# Autodesk Inventor assembly: POM_T5_31
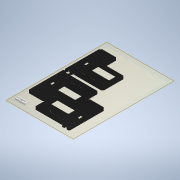
[picture p0: Inventor's stored thumbnail of the model, 180x180]
Saved by Autodesk Inventor 2020 (Build 240168000, 168)
## iProperties
Created: 2021-08-27
Part Number: POM_T5_31
Document SubType Name: Assembly
Designer: Masato
Author: Masato
## Documents named in this file (5)
- D:\GitHub\inventor\SUSTAINA-OP\Cam\POM_T5_31.iam
- D:\GitHub\inventor\SUSTAINA-OP\Cam\DisposableBoard.ipt
- D:\GitHub\inventor\SUSTAINA-OP\Jig\ForeArm_diagonal_Jig_2.ipt
- D:\GitHub\inventor\SUSTAINA-OP\UpperBody\Cockpit\Cockpit_side_frame.ipt
- D:\GitHub\inventor\SUSTAINA-OP\UpperBody\Cockpit\Cockpit_side_frame_MIR.ipt
## Components (5 placed, 4 different names)
1. DisposableBoard:1 — メイト:2, メイト:1, フラッシュ:1, フラッシュ:2, メイト:4, メイト:5, メイト:14, メイト:16, メイト:17, メイト:18, メイト:22, メイト:23, メイト:25
2. ForeArm_diagonal_Jig_2:1 — メイト:14, メイト:16, メイト:23
3. Cockpit_side_frame:1 — メイト:4, メイト:24, メイト:25
4. Cockpit_side_frame_MIR:2 — メイト:5, メイト:20, メイト:21, メイト:22, メイト:24
5. Cockpit_side_frame_MIR:3 — メイト:17, メイト:18, メイト:20, メイト:21
## Relationships (16: Mate 14, Flush 2)
- メイト:2 [Mate]: DisposableBoard:1
- メイト:1 [Mate]: DisposableBoard:1
- フラッシュ:1 [Flush]: DisposableBoard:1
- フラッシュ:2 [Flush]: DisposableBoard:1
- メイト:4 [Mate]: DisposableBoard:1 ↔ Cockpit_side_frame:1
- メイト:5 [Mate]: DisposableBoard:1 ↔ Cockpit_side_frame_MIR:2
- メイト:14 [Mate]: DisposableBoard:1 ↔ ForeArm_diagonal_Jig_2:1
- メイト:16 [Mate] (2 mm): DisposableBoard:1 ↔ ForeArm_diagonal_Jig_2:1
- メイト:17 [Mate]: DisposableBoard:1 ↔ Cockpit_side_frame_MIR:3
- メイト:18 [Mate] (2 mm): DisposableBoard:1 ↔ Cockpit_side_frame_MIR:3
- メイト:20 [Mate] (2.5 mm): Cockpit_side_frame_MIR:2 ↔ Cockpit_side_frame_MIR:3
- メイト:21 [Mate] (2.5 mm): Cockpit_side_frame_MIR:2 ↔ Cockpit_side_frame_MIR:3
- メイト:22 [Mate] (2 mm): DisposableBoard:1 ↔ Cockpit_side_frame_MIR:2
- メイト:23 [Mate] (2 mm): DisposableBoard:1 ↔ ForeArm_diagonal_Jig_2:1
- メイト:24 [Mate] (2.5 mm): Cockpit_side_frame:1 ↔ Cockpit_side_frame_MIR:2
- メイト:25 [Mate] (2 mm): DisposableBoard:1 ↔ Cockpit_side_frame:1
